# Autodesk Inventor assembly: CIM motor and shaft
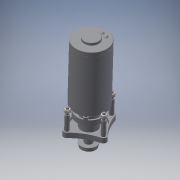
[picture p0: Inventor's stored thumbnail of the model, 180x180]
Saved by Autodesk Inventor 2019 (Build 230136000, 136)
## iProperties
Created: 2019-02-18
Part Number: CIM motor and shaft
Document SubType Name: Assembly
Designer: josh
Mass: 436.451 g
Surface Area: 763.411 cm^2
Volume: 434.057 cm^3
Density: 1.00551 g/cm^3
Author: josh
## Documents named in this file (3)
- D:\Synthesis Robots\Epsilon\Functioning swerve drive sub-assemblies\CIM motor and shaft.iam
- D:\Synthesis Robots\Epsilon\Functioning swerve drive sub-assemblies\Functioning swerve drive (CIM motor shaft).iam
- D:\Synthesis Robots\Epsilon\Functioning swerve drive sub-assemblies\Functioning swerve drive (motor).iam
## Components (2 placed, 2 different names)
1. Functioning swerve drive (CIM motor shaft):1 [sub-assembly] — Mate:1, Mate:2
2. Functioning swerve drive (motor):1 [sub-assembly] — Mate:1, Mate:2
## Relationships (2: Mate 2)
- Mate:1: Functioning swerve drive (CIM motor shaft):1 ↔ Functioning swerve drive (motor):1
- Mate:2 (4.7752 mm): Functioning swerve drive (CIM motor shaft):1 ↔ Functioning swerve drive (motor):1
